# Autodesk Inventor assembly: MCEN4000:M0
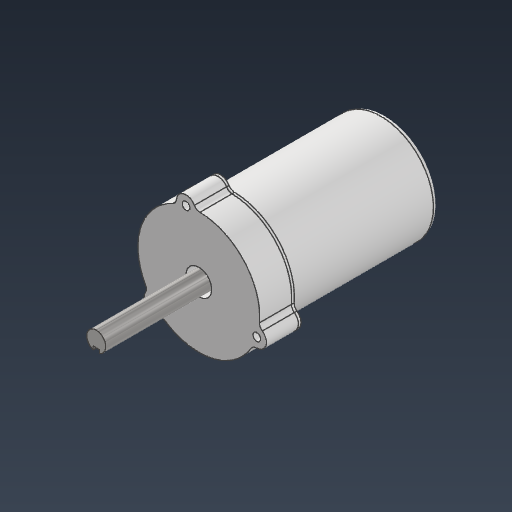
[picture p0: Inventor's stored thumbnail of the model, 512x512]
Saved by Autodesk Inventor 2021 (Build 250183000, 183)
## iProperties
Created: 2020-10-18
Part Number: MCEN4000:M0
Document SubType Name: Assembly
Designer: Eugene Tang
Mass: 718.887 g
Surface Area: 1404.85 cm^2
Volume: 718.887 cm^3
Density: 1 g/cm^3
Description: ELECTRI SERVO MOTOR
Author: Eugene Tang
## Documents named in this file (4)
- C:\Users\teuge\OneDrive - Curtin University of Technology Australia\Y4S2\DFM\Group Project\CAD\Parts\Assemblies\Motor Assembly.iam
- C:\Users\teuge\OneDrive - Curtin University of Technology Australia\Y4S2\DFM\Group Project\CAD\Parts\Motor Pin.ipt
- C:\Users\teuge\OneDrive - Curtin University of Technology Australia\Y4S2\DFM\Group Project\CAD\Parts\Motor Spacer.ipt
- C:\Users\teuge\OneDrive - Curtin University of Technology Australia\Y4S2\DFM\Group Project\CAD\Parts\Motor Cover.ipt
## Components (3 placed, 3 different names)
1. Motor Pin:1 — Mate:1, Mate:2, Mate:3
2. Motor Spacer:1 — Mate:1, Mate:2, Mate:4
3. Motor Cover:1 — Mate:3, Mate:4
## Relationships (4: Mate 4)
- Mate:1: Motor Pin:1 ↔ Motor Spacer:1
- Mate:2: Motor Pin:1 ↔ Motor Spacer:1
- Mate:3: Motor Pin:1 ↔ Motor Cover:1
- Mate:4: Motor Spacer:1 ↔ Motor Cover:1
